# Autodesk Inventor assembly: printer
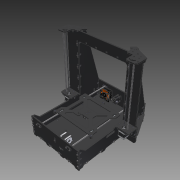
[picture p0: Inventor's stored thumbnail of the model, 180x180]
Saved by Autodesk Inventor 2014 (Build 180170000, 170)
## iProperties
Created: 2014-01-09
Part Number: printer
Document SubType Name: Assembly
Designer: buben
Author: buben
## Documents named in this file (40)
- C:\Users\buben\Documents\GitHub\bacon\inventor files\assemblies\printer.iam
- C:\Users\buben\Documents\GitHub\bacon\inventor files\printer parts\brace_left.ipt
- C:\Users\buben\Documents\GitHub\bacon\inventor files\printer parts\bottom.ipt
- C:\Users\buben\Documents\GitHub\bacon\inventor files\printer parts\brace_right.ipt
- C:\Users\buben\Documents\GitHub\bacon\inventor files\printer parts\front.ipt
- C:\Users\buben\Documents\GitHub\bacon\inventor files\printer parts\back.ipt
- C:\Users\buben\Documents\GitHub\bacon\inventor files\printer parts\frame.ipt
- C:\Users\buben\Documents\GitHub\bacon\inventor files\printer parts\z_motor_brace.ipt
- C:\Users\buben\Documents\GitHub\bacon\inventor files\printer parts\z_motor_mount.ipt
- C:\Users\buben\Documents\GitHub\bacon\inventor files\printer parts\y_axis_cap.ipt
- C:\Users\buben\Documents\GitHub\bacon\inventor files\printer parts\z_rod_stopper_bottom.ipt
- C:\Users\buben\Documents\GitHub\bacon\inventor files\3rd party components\nema_17_stepper\Imported Components\NEMA 17\NEMA 17.iam
- C:\Users\buben\Documents\GitHub\bacon\inventor files\utils\z_axis_rod.ipt
- C:\Users\buben\Documents\GitHub\bacon\inventor files\utils\z_threaded_rod.ipt
- C:\Users\buben\Documents\GitHub\bacon\inventor files\utils\y_axis_rod.ipt
- C:\Users\buben\Documents\GitHub\bacon\inventor files\printer parts\z_axis_top.ipt
- C:\Users\buben\Documents\GitHub\bacon\inventor files\printer parts\z_axis_top_cap.ipt
- C:\Users\buben\Documents\GitHub\bacon\inventor files\printer parts\frame_brace_top.ipt
- C:\Users\buben\Documents\GitHub\bacon\inventor files\utils\washer_m4.ipt
- C:\Users\buben\Documents\Inventor\Content Center Files\R2014\en-US\ISO 4762(2)\ISO 4762 - M4 x 20ISO.ipt
- C:\Users\buben\Documents\Inventor\Content Center Files\R2014\en-US\DIN 985\DIN 985 - M4.ipt
- C:\Users\buben\Documents\Inventor\Content Center Files\R2014\en-US\ISO 7040\ISO 7040 - M4.ipt
- C:\Users\buben\Documents\GitHub\bacon\inventor files\printer parts\wiring_brace.ipt
- C:\Users\buben\Documents\GitHub\bacon\inventor files\utils\washer_m3.ipt
- C:\Users\buben\Documents\Inventor\Content Center Files\R2014\en-US\ISO 4762(2)\ISO 4762 - M3 x 16ISO.ipt
- C:\Users\buben\Documents\GitHub\bacon\inventor files\3rd party components\PC Fan\Imported Components\PC Fan\PC Fan.iam
- C:\Users\buben\Documents\GitHub\bacon\inventor files\3rd party components\fan guard\Imported Components\User Library-Fan Guard\User Library-Fan Guard.ipt
- C:\Users\buben\Documents\GitHub\bacon\inventor files\printer parts\y_carriage_belt_iddler.ipt
- C:\Users\buben\Documents\GitHub\bacon\inventor files\printer parts\y_carriage_belt_iddler_holder.ipt
- C:\Users\buben\Documents\GitHub\bacon\inventor files\3rd party components\bearing_608\Imported Components\608RS\608RS.ipt
- C:\Users\buben\Documents\GitHub\bacon\inventor files\utils\belt_guide.ipt
- C:\Users\buben\Documents\GitHub\bacon\inventor files\utils\washer_m8.ipt
- C:\Users\buben\Documents\Inventor\Content Center Files\R2014\en-US\ISO 7040\ISO 7040 - M8.ipt
- C:\Users\buben\Documents\Inventor\Content Center Files\R2014\en-US\ISO 4762(2)\ISO 4762 - M8 x 40ISO.ipt
- C:\Users\buben\Documents\Inventor\Content Center Files\R2014\en-US\ISO 4762(2)\ISO 4762 - M4 x 30ISO.ipt
- C:\Users\buben\Documents\GitHub\bacon\inventor files\printer parts\y_motor_mount.ipt
- C:\Users\buben\Documents\GitHub\bacon\inventor files\printer parts\y_motor_mount_brace.ipt
- C:\Users\buben\Documents\GitHub\bacon\inventor files\printer parts\motor_spacer.ipt
- C:\Users\buben\Documents\GitHub\bacon\inventor files\3rd party components\nema_17_stepper\Imported Components\NEMA 17 with T5 Pulley\NEMA 17 with T5 Pulley.iam
- C:\Users\buben\Documents\GitHub\bacon\inventor files\assemblies\y_carryage.iam
## Components (360 placed, 39 different names)
1. brace_left:1 — Mate:1, Mate:2, Mate:3, Mate:4, Mate:5, Flush:1, Mate:8, Mate:9, Mate:10, Mate:11, Mate:13, Mate:14, Mate:15, Mate:16, Mate:23, Mate:24, Mate:25, Mate:78, Mate:79, Flush:3, Mate:123, Mate:205, Mate:207
2. bottom:1 — Mate:4, Mate:5, Flush:1, Mate:6, Flush:2, Mate:7, Mate:12, Mate:80, Mate:91
3. brace_right:1 — Mate:6, Flush:2, Mate:7, Mate:26, Mate:28, Mate:70, Mate:90, Mate:184, Mate:202, Mate:204, Mate:211, Mate:212
4. front:1 — Mate:8, Mate:9, Mate:10, Mate:29, Mate:30, Mate:31, Mate:32, Mate:33, Mate:34, Mate:84, Mate:85, Mate:86, Mate:87, Mate:134, Mate:135, Mate:304, Mate:305, Mate:306, Mate:307, Mate:308, Mate:309, Mate:310
5. back:1 — Mate:11, Mate:12, Mate:13, Mate:35, Mate:36, Mate:37, Mate:38, Mate:39, Mate:40, Insert:3, Insert:4, Mate:255, Mate:256, Mate:257, Mate:258, Mate:286, Mate:287, Mate:288, Mate:289, Mate:290, Mate:291, Mate:292
6. frame:1 — Mate:14, Mate:15, Mate:16, Mate:17, Mate:18, Mate:19, Mate:20, Mate:21, Mate:22, Mate:27, Mate:57, Mate:58, Mate:59, Mate:60, Mate:61, Mate:62, Mate:69, Mate:71, Flush:4, Mate:121, Mate:122, Mate:168, Mate:169, Mate:170, Mate:171, Mate:172, Mate:173, Mate:203, Mate:206, Mate:208, Mate:209
7. z_motor_brace:1 — Mate:20, Mate:21, Mate:22
8. z_motor_brace:2 — Mate:17, Mate:18, Mate:19, Mate:174, Mate:176
9. z_motor_mount:1 — Mate:23, Mate:24, Mate:25, Mate:44, Mate:45, Mate:46, Mate:52, Insert:2
10. z_motor_mount:2 — Mate:26, Mate:27, Mate:28, Mate:41, Mate:42, Mate:43, Insert:1, Mate:160, Mate:161, Mate:162, Mate:163, Mate:164, Mate:165, Mate:166, Mate:167, Mate:180, Mate:182, Mate:220, Mate:221, Mate:222, Mate:223, Mate:224, Mate:225, Mate:226, Mate:227
11. y_axis_cap:1 — Mate:30, Mate:33, Mate:34
12. y_axis_cap:2 — Mate:35, Mate:39, Mate:40
13. y_axis_cap:3 — Mate:36, Mate:37, Mate:38
14. y_axis_cap:4 — Mate:29, Mate:31, Mate:32, Mate:130, Mate:131, Mate:132, Mate:133
15. z_rod_stopper_bottom:1 — Mate:44, Mate:45, Mate:46, Mate:50, Mate:51
16. z_rod_stopper_bottom:2 — Mate:41, Mate:42, Mate:43, Mate:47, Mate:48, Mate:49, Mate:178, Mate:186
17. NEMA 17:1 [sub-assembly] — Mate:47, Mate:48, Mate:49, Mate:53, Mate:54
18. NEMA 17:2 [sub-assembly] — Mate:50, Mate:51, Mate:52, Mate:55, Mate:56
19. z_axis_rod:1 — Insert:1
20. z_axis_rod:2 — Insert:2
21. z_threaded_rod:1 — Mate:55, Mate:56
22. z_threaded_rod:2 — Mate:53, Mate:54
23. y_axis_rod:1 — Insert:3, Mate:338
24. y_axis_rod:2 — Insert:4, Mate:337
25. z_axis_top:1 — Mate:57, Mate:58, Mate:59, Mate:63, Mate:67, Mate:68
26. z_axis_top:2 — Mate:60, Mate:61, Mate:62, Mate:64, Mate:65, Mate:66
27. z_axis_top_cap:1 — Mate:63, Mate:67, Mate:68
28. z_axis_top_cap:2 — Mate:64, Mate:65, Mate:66
29. frame_brace_top:1 — Mate:69, Mate:70, Mate:71
30. DIN 985 - replaced by DIN EN ISO 10511 M4:12
31. CSN 02 1702 B B 4,3:30 — Insert:9
32. CSN 02 1702 B B 4,3:31 — Mate:106, Mate:108
33. ISO 4762 M4 x 20:15 — Mate:106, Insert:9, Mate:107
34. DIN EN ISO 7040 M4:6 — Mate:107, Mate:108
35. DIN EN ISO 7040 M4:7
36. CSN 02 1702 B B 4,3:32
37. ISO 4762 M4 x 20:16
38. CSN 02 1702 B B 4,3:33
39. DIN EN ISO 7040 M4:8
40. CSN 02 1702 B B 4,3:34
41. ISO 4762 M4 x 20:17
42. CSN 02 1702 B B 4,3:35
43. CSN 02 1702 B B 4,3:42 — Insert:10
44. CSN 02 1702 B B 4,3:43 — Insert:11
45. CSN 02 1702 B B 4,3:44 — Mate:109, Mate:112
46. CSN 02 1702 B B 4,3:45 — Mate:110, Mate:114
47. ISO 4762 M4 x 20:21 — Mate:109, Insert:10, Mate:111
48. ISO 4762 M4 x 20:22 — Mate:110, Insert:11, Mate:113
49. DIN EN ISO 7040 M4:12 — Mate:111, Mate:112
50. DIN EN ISO 7040 M4:13 — Mate:113, Mate:114
51. DIN EN ISO 7040 M4:14
52. CSN 02 1702 B B 4,3:46
53. ISO 4762 M4 x 20:23
54. CSN 02 1702 B B 4,3:47
55. DIN EN ISO 7040 M4:15
56. CSN 02 1702 B B 4,3:48
57. ISO 4762 M4 x 20:24
58. CSN 02 1702 B B 4,3:49
59. CSN 02 1702 B B 4,3:50 — Mate:115, Mate:116
60. ISO 4762 M4 x 20:25 — Mate:115, Mate:117
61. DIN EN ISO 7040 M4:16 — Mate:116, Mate:117
62. DIN EN ISO 7040 M4:17
63. CSN 02 1702 B B 4,3:51
64. ISO 4762 M4 x 20:26
65. CSN 02 1702 B B 4,3:52
66. DIN EN ISO 7040 M4:18
67. CSN 02 1702 B B 4,3:53
68. ISO 4762 M4 x 20:27
69. CSN 02 1702 B B 4,3:54
70. ISO 4762 M4 x 20:28
71. CSN 02 1702 B B 4,3:55
72. CSN 02 1702 B B 4,3:56
73. DIN EN ISO 7040 M4:19
74. ISO 4762 M4 x 20:29
75. CSN 02 1702 B B 4,3:57
76. CSN 02 1702 B B 4,3:58
77. DIN EN ISO 7040 M4:20
78. ISO 4762 M4 x 20:30
79. CSN 02 1702 B B 4,3:59
80. CSN 02 1702 B B 4,3:60
81. DIN EN ISO 7040 M4:21
82. ISO 4762 M4 x 20:35 — Mate:118, Insert:12, Mate:119
83. CSN 02 1702 B B 4,3:69 — Mate:118, Mate:120
84. CSN 02 1702 B B 4,3:70 — Insert:12
85. DIN EN ISO 7040 M4:26 — Mate:119, Mate:120
86. ISO 4762 M4 x 20:36
87. CSN 02 1702 B B 4,3:71
88. CSN 02 1702 B B 4,3:72
89. DIN EN ISO 7040 M4:27
90. ISO 4762 M4 x 20:37
91. CSN 02 1702 B B 4,3:73
92. CSN 02 1702 B B 4,3:74
93. DIN EN ISO 7040 M4:28
94. ISO 4762 M4 x 20:38
95. CSN 02 1702 B B 4,3:75
96. CSN 02 1702 B B 4,3:76
97. DIN EN ISO 7040 M4:29
98. ISO 4762 M4 x 20:39
99. CSN 02 1702 B B 4,3:77
100. CSN 02 1702 B B 4,3:78
101. DIN EN ISO 7040 M4:30
102. CSN 02 1702 B B 4,3:89 — Insert:14
103. CSN 02 1702 B B 4,3:90 — Mate:127, Mate:129
104. ISO 4762 M4 x 20:45 — Mate:127, Insert:14, Mate:128
105. DIN EN ISO 7040 M4:36 — Mate:128, Mate:129
106. ISO 4762 M4 x 20:46
107. CSN 02 1702 B B 4,3:91
108. CSN 02 1702 B B 4,3:92
109. DIN EN ISO 7040 M4:37
110. ISO 4762 M4 x 20:47
111. CSN 02 1702 B B 4,3:93
112. CSN 02 1702 B B 4,3:94
113. DIN EN ISO 7040 M4:38
114. ISO 4762 M4 x 20:48
115. CSN 02 1702 B B 4,3:95
116. CSN 02 1702 B B 4,3:96
117. DIN EN ISO 7040 M4:39
118. ISO 4762 M4 x 20:49
119. CSN 02 1702 B B 4,3:97
120. CSN 02 1702 B B 4,3:98
121. DIN EN ISO 7040 M4:40
122. CSN 02 1702 B B 4,3:99 — Mate:131, Mate:133, Insert:16
123. CSN 02 1702 B B 4,3:100 — Mate:130, Mate:132, Insert:15
124. CSN 02 1702 B B 4,3:101 — Mate:134, Mate:136, Mate:140
125. CSN 02 1702 B B 4,3:102 — Mate:135, Mate:137, Mate:138
126. ISO 4762 M4 x 20:50 — Insert:16, Mate:136, Mate:141
127. ISO 4762 M4 x 20:51 — Insert:15, Mate:137, Mate:139
128. DIN EN ISO 7040 M4:41 — Mate:138, Mate:139
129. DIN EN ISO 7040 M4:42 — Mate:140, Mate:141
130. CSN 02 1702 B B 4,3:103 — Insert:17
131. CSN 02 1702 B B 4,3:104 — Insert:18
132. CSN 02 1702 B B 4,3:105 — Mate:142, Mate:147
133. CSN 02 1702 B B 4,3:106 — Mate:143, Mate:145
134. ISO 4762 M4 x 20:52 — Mate:142, Insert:17, Mate:146
135. ISO 4762 M4 x 20:53 — Mate:143, Insert:18, Mate:144
136. DIN EN ISO 7040 M4:43 — Mate:144, Mate:145
137. DIN EN ISO 7040 M4:44 — Mate:146, Mate:147
138. CSN 02 1702 B B 4,3:107 — Insert:19
139. CSN 02 1702 B B 4,3:108 — Insert:20
140. CSN 02 1702 B B 4,3:109 — Mate:148, Mate:153
141. CSN 02 1702 B B 4,3:110 — Mate:149, Mate:151
142. ISO 4762 M4 x 20:54 — Mate:148, Insert:19, Mate:152
143. ISO 4762 M4 x 20:55 — Mate:149, Insert:20, Mate:150
144. DIN EN ISO 7040 M4:45 — Mate:150, Mate:151
145. DIN EN ISO 7040 M4:46 — Mate:152, Mate:153
146. CSN 02 1702 B B 4,3:111 — Insert:21
147. CSN 02 1702 B B 4,3:112 — Insert:22
148. CSN 02 1702 B B 4,3:113 — Mate:154, Mate:158
149. CSN 02 1702 B B 4,3:114 — Mate:155, Mate:156
150. ISO 4762 M4 x 20:56 — Insert:21, Mate:154, Mate:159
151. ISO 4762 M4 x 20:57 — Insert:22, Mate:155, Mate:157
152. DIN EN ISO 7040 M4:47 — Mate:156, Mate:157
153. DIN EN ISO 7040 M4:48 — Mate:158, Mate:159
154. CSN 02 1702 B B 4,3:115 — Mate:176, Mate:177, Mate:190
155. CSN 02 1702 B B 4,3:116 — Mate:164, Mate:165, Insert:25
156. CSN 02 1702 B B 4,3:117 — Mate:172, Mate:173, Insert:29
157. CSN 02 1702 B B 4,3:118 — Mate:182, Mate:183, Mate:196
158. CSN 02 1702 B B 4,3:119 — Mate:178, Mate:179, Mate:188
159. CSN 02 1702 B B 4,3:120 — Mate:162, Mate:163, Insert:23
160. CSN 02 1702 B B 4,3:121 — Mate:160, Mate:161, Insert:24
161. CSN 02 1702 B B 4,3:122 — Mate:166, Mate:167, Insert:26
162. CSN 02 1702 B B 4,3:123 — Mate:168, Mate:169, Insert:27
163. CSN 02 1702 B B 4,3:124 — Mate:170, Mate:171, Insert:28
164. CSN 02 1702 B B 4,3:125 — Mate:174, Mate:175, Mate:192
165. CSN 02 1702 B B 4,3:126 — Mate:184, Mate:185, Mate:198
166. CSN 02 1702 B B 4,3:127 — Mate:186, Mate:187, Mate:200
167. CSN 02 1702 B B 4,3:128 — Mate:180, Mate:181, Mate:194
168. ISO 4762 M4 x 20:58 — Insert:28, Mate:183, Mate:197
169. ISO 4762 M4 x 20:59 — Insert:29, Mate:175, Mate:193
170. ISO 4762 M4 x 20:60 — Insert:27, Mate:181, Mate:195
171. ISO 4762 M4 x 20:61 — Insert:26, Mate:187, Mate:201
172. ISO 4762 M4 x 20:62 — Insert:25, Mate:185, Mate:199
173. ISO 4762 M4 x 20:63 — Insert:24, Mate:179, Mate:189
174. ISO 4762 M4 x 20:64 — Insert:23, Mate:177, Mate:191
175. DIN EN ISO 7040 M4:49 — Mate:200, Mate:201
176. DIN EN ISO 7040 M4:50 — Mate:198, Mate:199
177. DIN EN ISO 7040 M4:51 — Mate:188, Mate:189
178. DIN EN ISO 7040 M4:52 — Mate:192, Mate:193
179. DIN EN ISO 7040 M4:53 — Mate:194, Mate:195
180. DIN EN ISO 7040 M4:54 — Mate:190, Mate:191
181. DIN EN ISO 7040 M4:55 — Mate:196, Mate:197
182. wiring_brace:1 — Mate:202, Mate:203, Mate:204, Mate:210, Mate:213
183. wiring_brace:2 — Mate:205, Mate:206, Mate:207
184. CSN 02 1702 B B 4,3:129 — Mate:211, Mate:212, Insert:31
185. CSN 02 1702 B B 4,3:130 — Mate:213, Mate:215, Mate:218
186. CSN 02 1702 B B 4,3:131 — Mate:210, Mate:214, Mate:216
187. CSN 02 1702 B B 4,3:132 — Mate:208, Mate:209, Insert:30
188. ISO 4762 M4 x 20:65 — Insert:30, Mate:214, Mate:217
189. ISO 4762 M4 x 20:66 — Insert:31, Mate:215, Mate:219
190. DIN EN ISO 7040 M4:56 — Mate:218, Mate:219
191. DIN EN ISO 7040 M4:57 — Mate:216, Mate:217
192. CSN 02 1702 B B 3,2:1 — Mate:222, Mate:227, Insert:35
193. CSN 02 1702 B B 3,2:2 — Mate:221, Mate:224, Insert:33
194. CSN 02 1702 B B 3,2:3 — Mate:220, Mate:226, Insert:34
195. CSN 02 1702 B B 3,2:4 — Mate:223, Mate:225, Insert:32
196. ISO 4762 M3 x 16:1 — Insert:33
197. ISO 4762 M3 x 16:2 — Insert:32
198. ISO 4762 M3 x 16:3 — Insert:34
199. ISO 4762 M3 x 16:4 — Insert:35
200. CSN 02 1702 B B 4,3:133 — Mate:234, Mate:246
201. CSN 02 1702 B B 4,3:134 — Insert:40
202. CSN 02 1702 B B 4,3:135 — Insert:37
203. CSN 02 1702 B B 4,3:136 — Mate:228, Mate:248
204. CSN 02 1702 B B 4,3:137 — Mate:233, Mate:240
205. CSN 02 1702 B B 4,3:138 — Insert:42
206. CSN 02 1702 B B 4,3:139 — Insert:41
207. CSN 02 1702 B B 4,3:140 — Insert:39
208. CSN 02 1702 B B 4,3:141 — Insert:38
209. CSN 02 1702 B B 4,3:142 — Insert:36
210. CSN 02 1702 B B 4,3:143 — Mate:229, Mate:242
211. CSN 02 1702 B B 4,3:144 — Mate:232, Mate:238
212. CSN 02 1702 B B 4,3:145 — Mate:231, Mate:236
213. CSN 02 1702 B B 4,3:146 — Mate:230, Mate:244
214. ISO 4762 M4 x 20:67 — Mate:228, Insert:36, Mate:247
215. ISO 4762 M4 x 20:68 — Mate:229, Insert:37, Mate:241
216. ISO 4762 M4 x 20:69 — Mate:230, Insert:38, Mate:243
217. ISO 4762 M4 x 20:70 — Mate:231, Insert:39, Mate:235
218. ISO 4762 M4 x 20:71 — Mate:232, Insert:40, Mate:237
219. ISO 4762 M4 x 20:72 — Mate:233, Insert:41, Mate:239
220. ISO 4762 M4 x 20:73 — Mate:234, Insert:42, Mate:245
221. DIN EN ISO 7040 M4:58 — Mate:235, Mate:236
222. DIN EN ISO 7040 M4:59 — Mate:237, Mate:238
223. DIN EN ISO 7040 M4:60 — Mate:239, Mate:240
224. DIN EN ISO 7040 M4:61 — Mate:241, Mate:242
225. DIN EN ISO 7040 M4:62 — Mate:243, Mate:244
226. DIN EN ISO 7040 M4:63 — Mate:245, Mate:246
227. DIN EN ISO 7040 M4:64 — Mate:247, Mate:248
228. CSN 02 1702 B B 4,3:147 — Insert:44
229. CSN 02 1702 B B 4,3:148 — Mate:250, Mate:252
230. CSN 02 1702 B B 4,3:149 — Mate:249, Mate:254
231. CSN 02 1702 B B 4,3:150 — Insert:43
232. ISO 4762 M4 x 20:74 — Mate:249, Insert:43, Mate:253
233. ISO 4762 M4 x 20:75 — Mate:250, Insert:44, Mate:251
234. DIN EN ISO 7040 M4:65 — Mate:251, Mate:252
235. DIN EN ISO 7040 M4:66 — Mate:253, Mate:254
236. CSN 02 1702 B B 3,2:5 — Insert:48
237. CSN 02 1702 B B 3,2:6 — Insert:45
238. CSN 02 1702 B B 3,2:7 — Insert:47
239. CSN 02 1702 B B 3,2:8 — Insert:46
240. ISO 4762 M3 x 16:5 — Insert:45
241. ISO 4762 M3 x 16:6 — Insert:46
242. ISO 4762 M3 x 16:7 — Insert:47
243. ISO 4762 M3 x 16:8 — Insert:48
244. PC Fan:1 [sub-assembly] — Mate:255, Mate:256, Mate:257
245. User Library-Fan Guard:1 — Mate:258
246. y_carriage_belt_iddler:1 — Mate:262, Mate:263, Mate:264, Mate:278, Mate:282, Mate:283, Mate:288
247. y_carriage_belt_iddler:2 — Mate:259, Mate:260, Mate:261, Mate:279, Mate:280, Mate:281, Mate:286, Mate:287
248. y_carriage_belt_iddler_holder:1 — Mate:259, Mate:260, Mate:261, Mate:262, Mate:263, Mate:264, Mate:293, Mate:294
249. 608RS:1 — Mate:265, Mate:266, Mate:269, Mate:274, Mate:275, Mate:276, Mate:277, Mate:279
250. belt_guide:1 — Mate:265, Mate:266, Mate:267, Mate:268
251. belt_guide:2 — Mate:267, Mate:268, Mate:269
252. CSN 02 1702 B B 8,4:1 — Mate:280, Mate:281, Mate:284
253. CSN 02 1702 B B 8,4:2 — Mate:282, Mate:283, Insert:49
254. CSN 02 1702 B B 8,4:3 — Mate:272, Mate:273
255. CSN 02 1702 B B 8,4:4 — Mate:272, Mate:273, Mate:274, Mate:275
256. CSN 02 1702 B B 8,4:5 — Mate:270, Mate:271, Mate:276, Mate:277
257. CSN 02 1702 B B 8,4:6 — Mate:270, Mate:271, Mate:278
258. ISO 4762 M8 x 40:1 — Insert:49, Mate:285
259. DIN EN ISO 7040 M8:1 — Mate:284, Mate:285
260. CSN 02 1702 B B 4,3:151 — Mate:294, Mate:295, Mate:297
261. CSN 02 1702 B B 4,3:152 — Mate:289, Mate:292, Insert:50
262. CSN 02 1702 B B 4,3:153 — Mate:290, Mate:291, Insert:51
263. CSN 02 1702 B B 4,3:154 — Mate:293, Mate:296, Mate:299
264. ISO 4762 M4 x 30:1 — Insert:50, Mate:296, Mate:300
265. ISO 4762 M4 x 30:2 — Insert:51, Mate:295, Mate:298
266. DIN EN ISO 7040 M4:67 — Mate:299, Mate:300
267. DIN EN ISO 7040 M4:68 — Mate:297, Mate:298
268. y_motor_mount:1 — Mate:301, Mate:302, Mate:303, Mate:304, Mate:306, Mate:311, Mate:312, Mate:317, Mate:328, Tangent:1, Tangent:2, Mate:329, Mate:330, Mate:331, Mate:332
269. y_motor_mount_brace:1 — Mate:301, Mate:302, Mate:303, Mate:305, Mate:313, Mate:315
270. CSN 02 1702 B B 4,3:155 — Mate:315, Mate:316, Mate:323
271. CSN 02 1702 B B 4,3:156 — Mate:317, Mate:318, Mate:319
272. CSN 02 1702 B B 4,3:157 — Mate:311, Mate:312, Insert:54
273. CSN 02 1702 B B 4,3:158 — Mate:313, Mate:314, Mate:321
274. CSN 02 1702 B B 4,3:159 — Mate:307, Mate:310, Insert:53
275. CSN 02 1702 B B 4,3:160 — Mate:308, Mate:309, Insert:52
276. ISO 4762 M4 x 20:76 — Insert:54, Mate:316, Mate:324
277. ISO 4762 M4 x 20:77 — Insert:53, Mate:318, Mate:320
278. ISO 4762 M4 x 20:78 — Insert:52, Mate:314, Mate:322
279. DIN EN ISO 7040 M4:69 — Mate:321, Mate:322
280. DIN EN ISO 7040 M4:70 — Mate:319, Mate:320
281. DIN EN ISO 7040 M4:71 — Mate:323, Mate:324
282. motor_spacer:1 — Mate:325, Mate:326, Mate:327, Mate:328, Tangent:1, Tangent:2, Mate:333, Mate:334, Mate:335, Mate:336
283. NEMA 17 with T5 Pulley:1 [sub-assembly] — Mate:325, Mate:326, Mate:327
284. CSN 02 1702 B B 3,2:9 — Mate:331, Insert:57
285. CSN 02 1702 B B 3,2:10 — Mate:332, Insert:58
286. CSN 02 1702 B B 3,2:11 — Mate:330, Insert:56
287. CSN 02 1702 B B 3,2:12 — Mate:329, Insert:55
288. ISO 4762 M3 x 16:9 — Insert:58, Mate:335
289. ISO 4762 M3 x 16:10 — Insert:57, Mate:336
290. ISO 4762 M3 x 16:11 — Insert:56, Mate:334
291. ISO 4762 M3 x 16:12 — Insert:55, Mate:333
292. y_carryage:1 [sub-assembly] — Mate:337, Mate:338
293. DIN EN ISO 7040 M4:2 — Mate:102, Mate:103
294. CSN 02 1702 B B 4,3:23 — Mate:90, Mate:94, Mate:102
295. ISO 4762 M4 x 20:11 — Insert:7, Mate:94, Mate:103
296. CSN 02 1702 B B 4,3:21 — Mate:84, Mate:85, Insert:7
297. DIN EN ISO 7040 M4:4
298. CSN 02 1702 B B 4,3:26
299. ISO 4762 M4 x 20:13
300. CSN 02 1702 B B 4,3:27
301. DIN EN ISO 7040 M4:5
302. CSN 02 1702 B B 4,3:28
303. ISO 4762 M4 x 20:14
304. CSN 02 1702 B B 4,3:29
305. ISO 4762 M4 x 20:12 — Insert:8, Mate:95, Mate:105
306. CSN 02 1702 B B 4,3:22 — Mate:86, Mate:87, Insert:8
307. CSN 02 1702 B B 4,3:25 — Mate:91, Mate:95, Mate:104
308. DIN EN ISO 7040 M4:3 — Mate:104, Mate:105
309. ISO 4762 M4 x 20:18
310. CSN 02 1702 B B 4,3:36
311. CSN 02 1702 B B 4,3:37
312. DIN EN ISO 7040 M4:9
313. ISO 4762 M4 x 20:19
314. CSN 02 1702 B B 4,3:38
315. CSN 02 1702 B B 4,3:39
316. DIN EN ISO 7040 M4:10
317. ISO 4762 M4 x 20:20
318. CSN 02 1702 B B 4,3:40
319. CSN 02 1702 B B 4,3:41
320. DIN EN ISO 7040 M4:11
321. ISO 4762 M4 x 20:6 — Insert:6, Mate:81, Mate:101
322. CSN 02 1702 B B 4,3:12 — Mate:78, Mate:79, Insert:6
323. CSN 02 1702 B B 4,3:11 — Mate:80, Mate:81, Mate:100
324. DIN EN ISO 7040 M4:1 — Mate:100, Mate:101
325. ISO 4762 M4 x 20:31
326. CSN 02 1702 B B 4,3:61
327. CSN 02 1702 B B 4,3:62
328. DIN EN ISO 7040 M4:22
329. ISO 4762 M4 x 20:32
330. CSN 02 1702 B B 4,3:63
331. CSN 02 1702 B B 4,3:64
332. DIN EN ISO 7040 M4:23
333. ISO 4762 M4 x 20:33
334. CSN 02 1702 B B 4,3:65
335. CSN 02 1702 B B 4,3:66
336. DIN EN ISO 7040 M4:24
337. ISO 4762 M4 x 20:34
338. CSN 02 1702 B B 4,3:67
339. CSN 02 1702 B B 4,3:68
340. DIN EN ISO 7040 M4:25
341. ISO 4762 M4 x 20:40 — Insert:13, Mate:124, Mate:126
342. CSN 02 1702 B B 4,3:79 — Mate:121, Mate:122, Insert:13
343. CSN 02 1702 B B 4,3:80 — Mate:123, Mate:124, Mate:125
344. DIN EN ISO 7040 M4:31 — Mate:125, Mate:126
345. ISO 4762 M4 x 20:41
346. CSN 02 1702 B B 4,3:81
347. CSN 02 1702 B B 4,3:82
348. DIN EN ISO 7040 M4:32
349. ISO 4762 M4 x 20:42
350. CSN 02 1702 B B 4,3:83
351. CSN 02 1702 B B 4,3:84
352. DIN EN ISO 7040 M4:33
353. ISO 4762 M4 x 20:43
354. CSN 02 1702 B B 4,3:85
355. CSN 02 1702 B B 4,3:86
356. DIN EN ISO 7040 M4:34
357. ISO 4762 M4 x 20:44
358. CSN 02 1702 B B 4,3:87
359. CSN 02 1702 B B 4,3:88
360. DIN EN ISO 7040 M4:35
## Component patterns: (3 elements, first: DIN EN ISO 7040 M4:2 + CSN 02 1702 B B 4,3:23 + ISO 4762 M4 x 20:11 + CSN 02 1702 B B 4,3:21), (4 elements, first: ISO 4762 M4 x 20:12 + CSN 02 1702 B B 4,3:22 + CSN 02 1702 B B 4,3:25 + DIN EN ISO 7040 M4:3), (5 elements, first: ISO 4762 M4 x 20:6 + CSN 02 1702 B B 4,3:12 + CSN 02 1702 B B 4,3:11 + DIN EN ISO 7040 M4:1), (5 elements, first: ISO 4762 M4 x 20:40 + CSN 02 1702 B B 4,3:79 + CSN 02 1702 B B 4,3:80 + DIN EN ISO 7040 M4:31)
## Relationships (385: Mate 322, Insert 57, Flush 4, Tangent 2)
- Mate:1: brace_left:1
- Mate:2: brace_left:1
- Mate:3: brace_left:1
- Mate:4: brace_left:1 ↔ bottom:1
- Mate:5: brace_left:1 ↔ bottom:1
- Flush:1: brace_left:1 ↔ bottom:1
- Mate:6: bottom:1 ↔ brace_right:1
- Flush:2: bottom:1 ↔ brace_right:1
- Mate:7: bottom:1 ↔ brace_right:1
- Mate:8: brace_left:1 ↔ front:1
- Mate:9: brace_left:1 ↔ front:1
- Mate:10: brace_left:1 ↔ front:1
- Mate:11: brace_left:1 ↔ back:1
- Mate:12: bottom:1 ↔ back:1
- Mate:13: brace_left:1 ↔ back:1
- Mate:14: brace_left:1 ↔ frame:1
- Mate:15: brace_left:1 ↔ frame:1
- Mate:16: brace_left:1 ↔ frame:1
- Mate:17: frame:1 ↔ z_motor_brace:2
- Mate:18: frame:1 ↔ z_motor_brace:2
- Mate:19: frame:1 ↔ z_motor_brace:2
- Mate:20: frame:1 ↔ z_motor_brace:1
- Mate:21: frame:1 ↔ z_motor_brace:1
- Mate:22: frame:1 ↔ z_motor_brace:1
- Mate:23: brace_left:1 ↔ z_motor_mount:1
- Mate:24: brace_left:1 ↔ z_motor_mount:1
- Mate:25: brace_left:1 ↔ z_motor_mount:1
- Mate:26: brace_right:1 ↔ z_motor_mount:2
- Mate:27: frame:1 ↔ z_motor_mount:2
- Mate:28: brace_right:1 ↔ z_motor_mount:2
- Mate:29: front:1 ↔ y_axis_cap:4
- Mate:30: front:1 ↔ y_axis_cap:1
- Mate:31: front:1 ↔ y_axis_cap:4
- Mate:32: front:1 ↔ y_axis_cap:4
- Mate:33: front:1 ↔ y_axis_cap:1
- Mate:34: front:1 ↔ y_axis_cap:1
- Mate:35: back:1 ↔ y_axis_cap:2
- Mate:36: back:1 ↔ y_axis_cap:3
- Mate:37: back:1 ↔ y_axis_cap:3
- Mate:38: back:1 ↔ y_axis_cap:3
- Mate:39: back:1 ↔ y_axis_cap:2
- Mate:40: back:1 ↔ y_axis_cap:2
- Mate:41: z_motor_mount:2 ↔ z_rod_stopper_bottom:2
- Mate:42: z_motor_mount:2 ↔ z_rod_stopper_bottom:2
- Mate:43: z_motor_mount:2 ↔ z_rod_stopper_bottom:2
- Mate:44: z_motor_mount:1 ↔ z_rod_stopper_bottom:1
- Mate:45: z_motor_mount:1 ↔ z_rod_stopper_bottom:1
- Mate:46: z_motor_mount:1 ↔ z_rod_stopper_bottom:1
- Mate:47: z_rod_stopper_bottom:2 ↔ NEMA 17:1
- Mate:48: z_rod_stopper_bottom:2 ↔ NEMA 17:1
- Mate:49: z_rod_stopper_bottom:2 ↔ NEMA 17:1
- Mate:50: z_rod_stopper_bottom:1 ↔ NEMA 17:2
- Mate:51: z_rod_stopper_bottom:1 ↔ NEMA 17:2
- Mate:52: z_motor_mount:1 ↔ NEMA 17:2
- Insert:1: z_motor_mount:2 ↔ z_axis_rod:1
- Insert:2: z_motor_mount:1 ↔ z_axis_rod:2
- Mate:53: NEMA 17:1 ↔ z_threaded_rod:2
- Mate:54: NEMA 17:1 ↔ z_threaded_rod:2
- Mate:55: NEMA 17:2 ↔ z_threaded_rod:1
- Mate:56: NEMA 17:2 ↔ z_threaded_rod:1
- Insert:3: back:1 ↔ y_axis_rod:1
- Insert:4: back:1 ↔ y_axis_rod:2
- Mate:57: frame:1 ↔ z_axis_top:1
- Mate:58: frame:1 ↔ z_axis_top:1
- Mate:59: frame:1 ↔ z_axis_top:1
- Mate:60: frame:1 ↔ z_axis_top:2
- Mate:61: frame:1 ↔ z_axis_top:2
- Mate:62: frame:1 ↔ z_axis_top:2
- Mate:63: z_axis_top:1 ↔ z_axis_top_cap:1
- Mate:64: z_axis_top:2 ↔ z_axis_top_cap:2
- Mate:65: z_axis_top:2 ↔ z_axis_top_cap:2
- Mate:66: z_axis_top:2 ↔ z_axis_top_cap:2
- Mate:67: z_axis_top:1 ↔ z_axis_top_cap:1
- Mate:68: z_axis_top:1 ↔ z_axis_top_cap:1
- Mate:69: frame:1 ↔ frame_brace_top:1
- Mate:70: brace_right:1 ↔ frame_brace_top:1
- Mate:71: frame:1 ↔ frame_brace_top:1
- Mate:78: brace_left:1 ↔ CSN 02 1702 B B 4,3:12
- Mate:79: brace_left:1 ↔ CSN 02 1702 B B 4,3:12
- Mate:80: bottom:1 ↔ CSN 02 1702 B B 4,3:11
- Insert:6: ISO 4762 M4 x 20:6 ↔ CSN 02 1702 B B 4,3:12
- Mate:81: ISO 4762 M4 x 20:6 ↔ CSN 02 1702 B B 4,3:11
- Mate:84: front:1 ↔ CSN 02 1702 B B 4,3:21
- Mate:85: front:1 ↔ CSN 02 1702 B B 4,3:21
- Mate:86: front:1 ↔ CSN 02 1702 B B 4,3:22
- Mate:87: front:1 ↔ CSN 02 1702 B B 4,3:22
- Mate:90: brace_right:1 ↔ CSN 02 1702 B B 4,3:23
- Mate:91: bottom:1 ↔ CSN 02 1702 B B 4,3:25
- Insert:7: ISO 4762 M4 x 20:11 ↔ CSN 02 1702 B B 4,3:21
- Insert:8: ISO 4762 M4 x 20:12 ↔ CSN 02 1702 B B 4,3:22
- Mate:94: CSN 02 1702 B B 4,3:23 ↔ ISO 4762 M4 x 20:11
- Mate:95: ISO 4762 M4 x 20:12 ↔ CSN 02 1702 B B 4,3:25
- Flush:3 (167.5 mm): brace_left:1
- Mate:100: CSN 02 1702 B B 4,3:11 ↔ DIN EN ISO 7040 M4:1
- Mate:101: ISO 4762 M4 x 20:6 ↔ DIN EN ISO 7040 M4:1
- Mate:102: DIN EN ISO 7040 M4:2 ↔ CSN 02 1702 B B 4,3:23
- Mate:103: DIN EN ISO 7040 M4:2 ↔ ISO 4762 M4 x 20:11
- Mate:104: CSN 02 1702 B B 4,3:25 ↔ DIN EN ISO 7040 M4:3
- Mate:105: ISO 4762 M4 x 20:12 ↔ DIN EN ISO 7040 M4:3
- Flush:4 (77 mm): frame:1
- Mate:106: CSN 02 1702 B B 4,3:31 ↔ ISO 4762 M4 x 20:15
- Insert:9: CSN 02 1702 B B 4,3:30 ↔ ISO 4762 M4 x 20:15
- Mate:107: ISO 4762 M4 x 20:15 ↔ DIN EN ISO 7040 M4:6
- Mate:108: CSN 02 1702 B B 4,3:31 ↔ DIN EN ISO 7040 M4:6
- Mate:109: CSN 02 1702 B B 4,3:44 ↔ ISO 4762 M4 x 20:21
- Insert:10: CSN 02 1702 B B 4,3:42 ↔ ISO 4762 M4 x 20:21
- Mate:110: CSN 02 1702 B B 4,3:45 ↔ ISO 4762 M4 x 20:22
- Insert:11: CSN 02 1702 B B 4,3:43 ↔ ISO 4762 M4 x 20:22
- Mate:111: ISO 4762 M4 x 20:21 ↔ DIN EN ISO 7040 M4:12
- Mate:112: CSN 02 1702 B B 4,3:44 ↔ DIN EN ISO 7040 M4:12
- Mate:113: ISO 4762 M4 x 20:22 ↔ DIN EN ISO 7040 M4:13
- Mate:114: CSN 02 1702 B B 4,3:45 ↔ DIN EN ISO 7040 M4:13
- Mate:115: CSN 02 1702 B B 4,3:50 ↔ ISO 4762 M4 x 20:25
- Mate:116: CSN 02 1702 B B 4,3:50 ↔ DIN EN ISO 7040 M4:16
- Mate:117: ISO 4762 M4 x 20:25 ↔ DIN EN ISO 7040 M4:16
- Mate:118: ISO 4762 M4 x 20:35 ↔ CSN 02 1702 B B 4,3:69
- Insert:12: ISO 4762 M4 x 20:35 ↔ CSN 02 1702 B B 4,3:70
- Mate:119: ISO 4762 M4 x 20:35 ↔ DIN EN ISO 7040 M4:26
- Mate:120: CSN 02 1702 B B 4,3:69 ↔ DIN EN ISO 7040 M4:26
- Mate:121: frame:1 ↔ CSN 02 1702 B B 4,3:79
- Mate:122: frame:1 ↔ CSN 02 1702 B B 4,3:79
- Insert:13: ISO 4762 M4 x 20:40 ↔ CSN 02 1702 B B 4,3:79
- Mate:123: brace_left:1 ↔ CSN 02 1702 B B 4,3:80
- Mate:124: ISO 4762 M4 x 20:40 ↔ CSN 02 1702 B B 4,3:80
- Mate:125: CSN 02 1702 B B 4,3:80 ↔ DIN EN ISO 7040 M4:31
- Mate:126: ISO 4762 M4 x 20:40 ↔ DIN EN ISO 7040 M4:31
- Mate:127: CSN 02 1702 B B 4,3:90 ↔ ISO 4762 M4 x 20:45
- Insert:14: CSN 02 1702 B B 4,3:89 ↔ ISO 4762 M4 x 20:45
- Mate:128: ISO 4762 M4 x 20:45 ↔ DIN EN ISO 7040 M4:36
- Mate:129: CSN 02 1702 B B 4,3:90 ↔ DIN EN ISO 7040 M4:36
- Mate:130: y_axis_cap:4 ↔ CSN 02 1702 B B 4,3:100
- Mate:131: y_axis_cap:4 ↔ CSN 02 1702 B B 4,3:99
- Mate:132: y_axis_cap:4 ↔ CSN 02 1702 B B 4,3:100
- Mate:133: y_axis_cap:4 ↔ CSN 02 1702 B B 4,3:99
- Mate:134: front:1 ↔ CSN 02 1702 B B 4,3:101
- Mate:135: front:1 ↔ CSN 02 1702 B B 4,3:102
- Insert:15: CSN 02 1702 B B 4,3:100 ↔ ISO 4762 M4 x 20:51
- Insert:16: CSN 02 1702 B B 4,3:99 ↔ ISO 4762 M4 x 20:50
- Mate:136: CSN 02 1702 B B 4,3:101 ↔ ISO 4762 M4 x 20:50
- Mate:137: CSN 02 1702 B B 4,3:102 ↔ ISO 4762 M4 x 20:51
- Mate:138: CSN 02 1702 B B 4,3:102 ↔ DIN EN ISO 7040 M4:41
- Mate:139: ISO 4762 M4 x 20:51 ↔ DIN EN ISO 7040 M4:41
- Mate:140: CSN 02 1702 B B 4,3:101 ↔ DIN EN ISO 7040 M4:42
- Mate:141: ISO 4762 M4 x 20:50 ↔ DIN EN ISO 7040 M4:42
- Mate:142: CSN 02 1702 B B 4,3:105 ↔ ISO 4762 M4 x 20:52
- Insert:17: CSN 02 1702 B B 4,3:103 ↔ ISO 4762 M4 x 20:52
- Mate:143: CSN 02 1702 B B 4,3:106 ↔ ISO 4762 M4 x 20:53
- Insert:18: CSN 02 1702 B B 4,3:104 ↔ ISO 4762 M4 x 20:53
- Mate:144: ISO 4762 M4 x 20:53 ↔ DIN EN ISO 7040 M4:43
- Mate:145: CSN 02 1702 B B 4,3:106 ↔ DIN EN ISO 7040 M4:43
- Mate:146: ISO 4762 M4 x 20:52 ↔ DIN EN ISO 7040 M4:44
- Mate:147: CSN 02 1702 B B 4,3:105 ↔ DIN EN ISO 7040 M4:44
- Mate:148: CSN 02 1702 B B 4,3:109 ↔ ISO 4762 M4 x 20:54
- Insert:19: CSN 02 1702 B B 4,3:107 ↔ ISO 4762 M4 x 20:54
- Mate:149: CSN 02 1702 B B 4,3:110 ↔ ISO 4762 M4 x 20:55
- Insert:20: CSN 02 1702 B B 4,3:108 ↔ ISO 4762 M4 x 20:55
- Mate:150: ISO 4762 M4 x 20:55 ↔ DIN EN ISO 7040 M4:45
- Mate:151: CSN 02 1702 B B 4,3:110 ↔ DIN EN ISO 7040 M4:45
- Mate:152: ISO 4762 M4 x 20:54 ↔ DIN EN ISO 7040 M4:46
- Mate:153: CSN 02 1702 B B 4,3:109 ↔ DIN EN ISO 7040 M4:46
- Insert:21: CSN 02 1702 B B 4,3:111 ↔ ISO 4762 M4 x 20:56
- Mate:154: CSN 02 1702 B B 4,3:113 ↔ ISO 4762 M4 x 20:56
- Insert:22: CSN 02 1702 B B 4,3:112 ↔ ISO 4762 M4 x 20:57
- Mate:155: CSN 02 1702 B B 4,3:114 ↔ ISO 4762 M4 x 20:57
- Mate:156: CSN 02 1702 B B 4,3:114 ↔ DIN EN ISO 7040 M4:47
- Mate:157: ISO 4762 M4 x 20:57 ↔ DIN EN ISO 7040 M4:47
- Mate:158: CSN 02 1702 B B 4,3:113 ↔ DIN EN ISO 7040 M4:48
- Mate:159: ISO 4762 M4 x 20:56 ↔ DIN EN ISO 7040 M4:48
- Mate:160: z_motor_mount:2 ↔ CSN 02 1702 B B 4,3:121
- Mate:161: z_motor_mount:2 ↔ CSN 02 1702 B B 4,3:121
- Mate:162: z_motor_mount:2 ↔ CSN 02 1702 B B 4,3:120
- Mate:163: z_motor_mount:2 ↔ CSN 02 1702 B B 4,3:120
- Mate:164: z_motor_mount:2 ↔ CSN 02 1702 B B 4,3:116
- Mate:165: z_motor_mount:2 ↔ CSN 02 1702 B B 4,3:116
- Mate:166: z_motor_mount:2 ↔ CSN 02 1702 B B 4,3:122
- Mate:167: z_motor_mount:2 ↔ CSN 02 1702 B B 4,3:122
- Mate:168: frame:1 ↔ CSN 02 1702 B B 4,3:123
- Mate:169: frame:1 ↔ CSN 02 1702 B B 4,3:123
- Mate:170: frame:1 ↔ CSN 02 1702 B B 4,3:124
- Mate:171: frame:1 ↔ CSN 02 1702 B B 4,3:124
- Mate:172: frame:1 ↔ CSN 02 1702 B B 4,3:117
- Mate:173: frame:1 ↔ CSN 02 1702 B B 4,3:117
- Insert:23: CSN 02 1702 B B 4,3:120 ↔ ISO 4762 M4 x 20:64
- Insert:24: CSN 02 1702 B B 4,3:121 ↔ ISO 4762 M4 x 20:63
- Insert:25: CSN 02 1702 B B 4,3:116 ↔ ISO 4762 M4 x 20:62
- Insert:26: CSN 02 1702 B B 4,3:122 ↔ ISO 4762 M4 x 20:61
- Insert:27: CSN 02 1702 B B 4,3:123 ↔ ISO 4762 M4 x 20:60
- Insert:28: CSN 02 1702 B B 4,3:124 ↔ ISO 4762 M4 x 20:58
- Insert:29: CSN 02 1702 B B 4,3:117 ↔ ISO 4762 M4 x 20:59
- Mate:174: z_motor_brace:2 ↔ CSN 02 1702 B B 4,3:125
- Mate:175: CSN 02 1702 B B 4,3:125 ↔ ISO 4762 M4 x 20:59
- Mate:176: z_motor_brace:2 ↔ CSN 02 1702 B B 4,3:115
- Mate:177: CSN 02 1702 B B 4,3:115 ↔ ISO 4762 M4 x 20:64
- Mate:178: z_rod_stopper_bottom:2 ↔ CSN 02 1702 B B 4,3:119
- Mate:179: CSN 02 1702 B B 4,3:119 ↔ ISO 4762 M4 x 20:63
- Mate:180: z_motor_mount:2 ↔ CSN 02 1702 B B 4,3:128
- Mate:181: CSN 02 1702 B B 4,3:128 ↔ ISO 4762 M4 x 20:60
- Mate:182: z_motor_mount:2 ↔ CSN 02 1702 B B 4,3:118
- Mate:183: CSN 02 1702 B B 4,3:118 ↔ ISO 4762 M4 x 20:58
- Mate:184: brace_right:1 ↔ CSN 02 1702 B B 4,3:126
- Mate:185: CSN 02 1702 B B 4,3:126 ↔ ISO 4762 M4 x 20:62
- Mate:186: z_rod_stopper_bottom:2 ↔ CSN 02 1702 B B 4,3:127
- Mate:187: CSN 02 1702 B B 4,3:127 ↔ ISO 4762 M4 x 20:61
- Mate:188: CSN 02 1702 B B 4,3:119 ↔ DIN EN ISO 7040 M4:51
- Mate:189: ISO 4762 M4 x 20:63 ↔ DIN EN ISO 7040 M4:51
- Mate:190: CSN 02 1702 B B 4,3:115 ↔ DIN EN ISO 7040 M4:54
- Mate:191: ISO 4762 M4 x 20:64 ↔ DIN EN ISO 7040 M4:54
- Mate:192: CSN 02 1702 B B 4,3:125 ↔ DIN EN ISO 7040 M4:52
- Mate:193: ISO 4762 M4 x 20:59 ↔ DIN EN ISO 7040 M4:52
- Mate:194: CSN 02 1702 B B 4,3:128 ↔ DIN EN ISO 7040 M4:53
- Mate:195: ISO 4762 M4 x 20:60 ↔ DIN EN ISO 7040 M4:53
- Mate:196: CSN 02 1702 B B 4,3:118 ↔ DIN EN ISO 7040 M4:55
- Mate:197: ISO 4762 M4 x 20:58 ↔ DIN EN ISO 7040 M4:55
- Mate:198: CSN 02 1702 B B 4,3:126 ↔ DIN EN ISO 7040 M4:50
- Mate:199: ISO 4762 M4 x 20:62 ↔ DIN EN ISO 7040 M4:50
- Mate:200: CSN 02 1702 B B 4,3:127 ↔ DIN EN ISO 7040 M4:49
- Mate:201: ISO 4762 M4 x 20:61 ↔ DIN EN ISO 7040 M4:49
- Mate:202: brace_right:1 ↔ wiring_brace:1
- Mate:203: frame:1 ↔ wiring_brace:1
- Mate:204: brace_right:1 ↔ wiring_brace:1
- Mate:205: brace_left:1 ↔ wiring_brace:2
- Mate:206: frame:1 ↔ wiring_brace:2
- Mate:207: brace_left:1 ↔ wiring_brace:2
- Mate:208: frame:1 ↔ CSN 02 1702 B B 4,3:132
- Mate:209: frame:1 ↔ CSN 02 1702 B B 4,3:132
- Mate:210: wiring_brace:1 ↔ CSN 02 1702 B B 4,3:131
- Mate:211: brace_right:1 ↔ CSN 02 1702 B B 4,3:129
- Mate:212: brace_right:1 ↔ CSN 02 1702 B B 4,3:129
- Mate:213: wiring_brace:1 ↔ CSN 02 1702 B B 4,3:130
- Insert:30: CSN 02 1702 B B 4,3:132 ↔ ISO 4762 M4 x 20:65
- Insert:31: CSN 02 1702 B B 4,3:129 ↔ ISO 4762 M4 x 20:66
- Mate:214: CSN 02 1702 B B 4,3:131 ↔ ISO 4762 M4 x 20:65
- Mate:215: CSN 02 1702 B B 4,3:130 ↔ ISO 4762 M4 x 20:66
- Mate:216: CSN 02 1702 B B 4,3:131 ↔ DIN EN ISO 7040 M4:57
- Mate:217: ISO 4762 M4 x 20:65 ↔ DIN EN ISO 7040 M4:57
- Mate:218: CSN 02 1702 B B 4,3:130 ↔ DIN EN ISO 7040 M4:56
- Mate:219: ISO 4762 M4 x 20:66 ↔ DIN EN ISO 7040 M4:56
- Mate:220: z_motor_mount:2 ↔ CSN 02 1702 B B 3,2:3
- Mate:221: z_motor_mount:2 ↔ CSN 02 1702 B B 3,2:2
- Mate:222: z_motor_mount:2 ↔ CSN 02 1702 B B 3,2:1
- Mate:223: z_motor_mount:2 ↔ CSN 02 1702 B B 3,2:4
- Mate:224: z_motor_mount:2 ↔ CSN 02 1702 B B 3,2:2
- Mate:225: z_motor_mount:2 ↔ CSN 02 1702 B B 3,2:4
- Mate:226: z_motor_mount:2 ↔ CSN 02 1702 B B 3,2:3
- Mate:227: z_motor_mount:2 ↔ CSN 02 1702 B B 3,2:1
- Insert:32: CSN 02 1702 B B 3,2:4 ↔ ISO 4762 M3 x 16:2
- Insert:33: CSN 02 1702 B B 3,2:2 ↔ ISO 4762 M3 x 16:1
- Insert:34: CSN 02 1702 B B 3,2:3 ↔ ISO 4762 M3 x 16:3
- Insert:35: CSN 02 1702 B B 3,2:1 ↔ ISO 4762 M3 x 16:4
- Mate:228: CSN 02 1702 B B 4,3:136 ↔ ISO 4762 M4 x 20:67
- Insert:36: CSN 02 1702 B B 4,3:142 ↔ ISO 4762 M4 x 20:67
- Mate:229: CSN 02 1702 B B 4,3:143 ↔ ISO 4762 M4 x 20:68
- Insert:37: CSN 02 1702 B B 4,3:135 ↔ ISO 4762 M4 x 20:68
- Mate:230: CSN 02 1702 B B 4,3:146 ↔ ISO 4762 M4 x 20:69
- Insert:38: CSN 02 1702 B B 4,3:141 ↔ ISO 4762 M4 x 20:69
- Mate:231: CSN 02 1702 B B 4,3:145 ↔ ISO 4762 M4 x 20:70
- Insert:39: CSN 02 1702 B B 4,3:140 ↔ ISO 4762 M4 x 20:70
- Mate:232: CSN 02 1702 B B 4,3:144 ↔ ISO 4762 M4 x 20:71
- Insert:40: CSN 02 1702 B B 4,3:134 ↔ ISO 4762 M4 x 20:71
- Mate:233: CSN 02 1702 B B 4,3:137 ↔ ISO 4762 M4 x 20:72
- Insert:41: CSN 02 1702 B B 4,3:139 ↔ ISO 4762 M4 x 20:72
- Mate:234: CSN 02 1702 B B 4,3:133 ↔ ISO 4762 M4 x 20:73
- Insert:42: CSN 02 1702 B B 4,3:138 ↔ ISO 4762 M4 x 20:73
- Mate:235: ISO 4762 M4 x 20:70 ↔ DIN EN ISO 7040 M4:58
- Mate:236: CSN 02 1702 B B 4,3:145 ↔ DIN EN ISO 7040 M4:58
- Mate:237: ISO 4762 M4 x 20:71 ↔ DIN EN ISO 7040 M4:59
- Mate:238: CSN 02 1702 B B 4,3:144 ↔ DIN EN ISO 7040 M4:59
- Mate:239: ISO 4762 M4 x 20:72 ↔ DIN EN ISO 7040 M4:60
- Mate:240: CSN 02 1702 B B 4,3:137 ↔ DIN EN ISO 7040 M4:60
- Mate:241: ISO 4762 M4 x 20:68 ↔ DIN EN ISO 7040 M4:61
- Mate:242: CSN 02 1702 B B 4,3:143 ↔ DIN EN ISO 7040 M4:61
- Mate:243: ISO 4762 M4 x 20:69 ↔ DIN EN ISO 7040 M4:62
- Mate:244: CSN 02 1702 B B 4,3:146 ↔ DIN EN ISO 7040 M4:62
- Mate:245: ISO 4762 M4 x 20:73 ↔ DIN EN ISO 7040 M4:63
- Mate:246: CSN 02 1702 B B 4,3:133 ↔ DIN EN ISO 7040 M4:63
- Mate:247: ISO 4762 M4 x 20:67 ↔ DIN EN ISO 7040 M4:64
- Mate:248: CSN 02 1702 B B 4,3:136 ↔ DIN EN ISO 7040 M4:64
- Mate:249: CSN 02 1702 B B 4,3:149 ↔ ISO 4762 M4 x 20:74
- Insert:43: CSN 02 1702 B B 4,3:150 ↔ ISO 4762 M4 x 20:74
- Mate:250: CSN 02 1702 B B 4,3:148 ↔ ISO 4762 M4 x 20:75
- Insert:44: CSN 02 1702 B B 4,3:147 ↔ ISO 4762 M4 x 20:75
- Mate:251: ISO 4762 M4 x 20:75 ↔ DIN EN ISO 7040 M4:65
- Mate:252: CSN 02 1702 B B 4,3:148 ↔ DIN EN ISO 7040 M4:65
- Mate:253: ISO 4762 M4 x 20:74 ↔ DIN EN ISO 7040 M4:66
- Mate:254: CSN 02 1702 B B 4,3:149 ↔ DIN EN ISO 7040 M4:66
- Insert:45: CSN 02 1702 B B 3,2:6 ↔ ISO 4762 M3 x 16:5
- Insert:46: CSN 02 1702 B B 3,2:8 ↔ ISO 4762 M3 x 16:6
- Insert:47: CSN 02 1702 B B 3,2:7 ↔ ISO 4762 M3 x 16:7
- Insert:48: CSN 02 1702 B B 3,2:5 ↔ ISO 4762 M3 x 16:8
- Mate:255: back:1 ↔ PC Fan:1
- Mate:256: back:1 ↔ PC Fan:1
- Mate:257: back:1 ↔ PC Fan:1
- Mate:258 (3 mm): back:1 ↔ User Library-Fan Guard:1
- Mate:259: y_carriage_belt_iddler:2 ↔ y_carriage_belt_iddler_holder:1
- Mate:260: y_carriage_belt_iddler:2 ↔ y_carriage_belt_iddler_holder:1
- Mate:261: y_carriage_belt_iddler:2 ↔ y_carriage_belt_iddler_holder:1
- Mate:262: y_carriage_belt_iddler:1 ↔ y_carriage_belt_iddler_holder:1
- Mate:263: y_carriage_belt_iddler:1 ↔ y_carriage_belt_iddler_holder:1
- Mate:264: y_carriage_belt_iddler:1 ↔ y_carriage_belt_iddler_holder:1
- Mate:265: 608RS:1 ↔ belt_guide:1
- Mate:266: 608RS:1 ↔ belt_guide:1
- Mate:267: belt_guide:1 ↔ belt_guide:2
- Mate:268: belt_guide:1 ↔ belt_guide:2
- Mate:269: 608RS:1 ↔ belt_guide:2
- Mate:270: CSN 02 1702 B B 8,4:5 ↔ CSN 02 1702 B B 8,4:6
- Mate:271: CSN 02 1702 B B 8,4:5 ↔ CSN 02 1702 B B 8,4:6
- Mate:272: CSN 02 1702 B B 8,4:3 ↔ CSN 02 1702 B B 8,4:4
- Mate:273: CSN 02 1702 B B 8,4:3 ↔ CSN 02 1702 B B 8,4:4
- Mate:274: 608RS:1 ↔ CSN 02 1702 B B 8,4:4
- Mate:275: 608RS:1 ↔ CSN 02 1702 B B 8,4:4
- Mate:276: 608RS:1 ↔ CSN 02 1702 B B 8,4:5
- Mate:277: 608RS:1 ↔ CSN 02 1702 B B 8,4:5
- Mate:278: y_carriage_belt_iddler:1 ↔ CSN 02 1702 B B 8,4:6
- Mate:279: y_carriage_belt_iddler:2 ↔ 608RS:1
- Mate:280: y_carriage_belt_iddler:2 ↔ CSN 02 1702 B B 8,4:1
- Mate:281: y_carriage_belt_iddler:2 ↔ CSN 02 1702 B B 8,4:1
- Mate:282: y_carriage_belt_iddler:1 ↔ CSN 02 1702 B B 8,4:2
- Mate:283: y_carriage_belt_iddler:1 ↔ CSN 02 1702 B B 8,4:2
- Insert:49: CSN 02 1702 B B 8,4:2 ↔ ISO 4762 M8 x 40:1
- Mate:284: CSN 02 1702 B B 8,4:1 ↔ DIN EN ISO 7040 M8:1
- Mate:285: ISO 4762 M8 x 40:1 ↔ DIN EN ISO 7040 M8:1
- Mate:286: back:1 ↔ y_carriage_belt_iddler:2
- Mate:287: back:1 ↔ y_carriage_belt_iddler:2
- Mate:288: back:1 ↔ y_carriage_belt_iddler:1
- Mate:289: back:1 ↔ CSN 02 1702 B B 4,3:152
- Mate:290: back:1 ↔ CSN 02 1702 B B 4,3:153
- Mate:291: back:1 ↔ CSN 02 1702 B B 4,3:153
- Mate:292: back:1 ↔ CSN 02 1702 B B 4,3:152
- Insert:50: CSN 02 1702 B B 4,3:152 ↔ ISO 4762 M4 x 30:1
- Insert:51: CSN 02 1702 B B 4,3:153 ↔ ISO 4762 M4 x 30:2
- Mate:293: y_carriage_belt_iddler_holder:1 ↔ CSN 02 1702 B B 4,3:154
- Mate:294: y_carriage_belt_iddler_holder:1 ↔ CSN 02 1702 B B 4,3:151
- Mate:295: CSN 02 1702 B B 4,3:151 ↔ ISO 4762 M4 x 30:2
- Mate:296: CSN 02 1702 B B 4,3:154 ↔ ISO 4762 M4 x 30:1
- Mate:297: CSN 02 1702 B B 4,3:151 ↔ DIN EN ISO 7040 M4:68
- Mate:298: ISO 4762 M4 x 30:2 ↔ DIN EN ISO 7040 M4:68
- Mate:299: CSN 02 1702 B B 4,3:154 ↔ DIN EN ISO 7040 M4:67
- Mate:300: ISO 4762 M4 x 30:1 ↔ DIN EN ISO 7040 M4:67
- Mate:301: y_motor_mount:1 ↔ y_motor_mount_brace:1
- Mate:302: y_motor_mount:1 ↔ y_motor_mount_brace:1
- Mate:303: y_motor_mount:1 ↔ y_motor_mount_brace:1
- Mate:304: front:1 ↔ y_motor_mount:1
- Mate:305: front:1 ↔ y_motor_mount_brace:1
- Mate:306: front:1 ↔ y_motor_mount:1
- Mate:307: front:1 ↔ CSN 02 1702 B B 4,3:159
- Mate:308: front:1 ↔ CSN 02 1702 B B 4,3:160
- Mate:309: front:1 ↔ CSN 02 1702 B B 4,3:160
- Mate:310: front:1 ↔ CSN 02 1702 B B 4,3:159
- Mate:311: y_motor_mount:1 ↔ CSN 02 1702 B B 4,3:157
- Mate:312: y_motor_mount:1 ↔ CSN 02 1702 B B 4,3:157
- Insert:52: CSN 02 1702 B B 4,3:160 ↔ ISO 4762 M4 x 20:78
- Insert:53: CSN 02 1702 B B 4,3:159 ↔ ISO 4762 M4 x 20:77
- Insert:54: CSN 02 1702 B B 4,3:157 ↔ ISO 4762 M4 x 20:76
- Mate:313: y_motor_mount_brace:1 ↔ CSN 02 1702 B B 4,3:158
- Mate:314: CSN 02 1702 B B 4,3:158 ↔ ISO 4762 M4 x 20:78
- Mate:315: y_motor_mount_brace:1 ↔ CSN 02 1702 B B 4,3:155
- Mate:316: CSN 02 1702 B B 4,3:155 ↔ ISO 4762 M4 x 20:76
- Mate:317: y_motor_mount:1 ↔ CSN 02 1702 B B 4,3:156
- Mate:318: CSN 02 1702 B B 4,3:156 ↔ ISO 4762 M4 x 20:77
- Mate:319: CSN 02 1702 B B 4,3:156 ↔ DIN EN ISO 7040 M4:70
- Mate:320: ISO 4762 M4 x 20:77 ↔ DIN EN ISO 7040 M4:70
- Mate:321: CSN 02 1702 B B 4,3:158 ↔ DIN EN ISO 7040 M4:69
- Mate:322: ISO 4762 M4 x 20:78 ↔ DIN EN ISO 7040 M4:69
- Mate:323: CSN 02 1702 B B 4,3:155 ↔ DIN EN ISO 7040 M4:71
- Mate:324: ISO 4762 M4 x 20:76 ↔ DIN EN ISO 7040 M4:71
- Mate:325: motor_spacer:1 ↔ NEMA 17 with T5 Pulley:1
- Mate:326: motor_spacer:1 ↔ NEMA 17 with T5 Pulley:1
- Mate:327: motor_spacer:1 ↔ NEMA 17 with T5 Pulley:1
- Mate:328: y_motor_mount:1 ↔ motor_spacer:1
- Tangent:1: y_motor_mount:1 ↔ motor_spacer:1
- Tangent:2: y_motor_mount:1 ↔ motor_spacer:1
- Mate:329: y_motor_mount:1 ↔ CSN 02 1702 B B 3,2:12
- Mate:330: y_motor_mount:1 ↔ CSN 02 1702 B B 3,2:11
- Mate:331: y_motor_mount:1 ↔ CSN 02 1702 B B 3,2:9
- Mate:332: y_motor_mount:1 ↔ CSN 02 1702 B B 3,2:10
- Insert:55: CSN 02 1702 B B 3,2:12 ↔ ISO 4762 M3 x 16:12
- Insert:56: CSN 02 1702 B B 3,2:11 ↔ ISO 4762 M3 x 16:11
- Insert:57: CSN 02 1702 B B 3,2:9 ↔ ISO 4762 M3 x 16:10
- Insert:58: CSN 02 1702 B B 3,2:10 ↔ ISO 4762 M3 x 16:9
- Mate:333: motor_spacer:1 ↔ ISO 4762 M3 x 16:12
- Mate:334: motor_spacer:1 ↔ ISO 4762 M3 x 16:11
- Mate:335: motor_spacer:1 ↔ ISO 4762 M3 x 16:9
- Mate:336: motor_spacer:1 ↔ ISO 4762 M3 x 16:10
- Mate:337: y_axis_rod:2 ↔ y_carryage:1
- Mate:338: y_axis_rod:1 ↔ y_carryage:1
